# Autodesk Inventor assembly: Robot
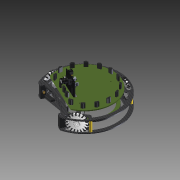
[picture p0: Inventor's stored thumbnail of the model, 180x180]
Saved by Autodesk Inventor 2015 (Build 190159000, 159)
## iProperties
Created: 2016-08-02
Part Number: Robot
Document SubType Name: Assembly
Designer: James Yelland
Author: James Yelland
## Documents named in this file (14)
- C:\Users\James Yelland\git\Layers-2017\Models\Robot.iam
- C:\Users\James Yelland\git\Layers-2017\Models\Bottom Plate.ipt
- C:\Users\James Yelland\git\Layers-2017\Models\Motor Mount.ipt
- C:\Users\James Yelland\git\Layers-2017\Models\Standoff 30.ipt
- C:\Users\James Yelland\git\Layers-2017\Models\Motor.ipt
- C:\Users\James Yelland\git\Layers-2017\Models\Middle Plate.ipt
- C:\Users\James Yelland\git\Layers-2017\Models\PCB.ipt
- C:\Users\James Yelland\git\Layers-2017\Models\Standoff 10.ipt
- C:\Users\James Yelland\git\Layers-2017\Models\Imported Components\Pixy(CMUcam5)\Pixy(CMUcam5).iam
- C:\Users\James Yelland\git\Layers-2017\Models\Light Sensor PCB.ipt
- C:\Users\James Yelland\git\Layers-2017\Models\Solenoid Mount.ipt
- C:\Users\James Yelland\git\Layers-2017\Models\Wheel.ipt
- C:\Users\James Yelland\git\Layers-2017\Models\Kicker Plate.ipt
- C:\Users\James Yelland\git\Layers-2017\Models\Laser Diode.ipt
## Components (24 placed, 13 different names)
1. Bottom Plate:1 — Mate:1, Mate:2, Mate:3, Mate:4, Mate:5, Mate:6, Mate:7, Mate:8, Mate:9, Mate:57, Mate:73, Mate:74, Mate:75, Mate:76, Mate:77, Mate:78, Mate:79, Mate:80, Mate:88, Mate:89, Mate:90, Flush:9, Flush:10
2. Motor Mount:1 — Mate:1, Mate:2, Mate:6, Mate:24, Mate:25, Mate:26
3. Motor Mount:2 — Mate:3, Mate:4, Mate:5, Mate:23, Mate:27, Mate:28
4. Motor Mount:3 — Mate:7, Mate:8, Mate:9, Mate:22, Mate:29, Mate:30
5. Motor:1 — Mate:24, Mate:25, Mate:26, Mate:91, Flush:7
6. Motor:2 — Mate:23, Mate:27, Mate:28, Mate:92, Flush:8
7. Motor:3 — Mate:22, Mate:29, Mate:30, Mate:93, Flush:6
8. Middle Plate:1 — Mate:37, Mate:38, Mate:39, Mate:40, Mate:41, Mate:42, Mate:87, Mate:94, Mate:98
9. PCB:1 — Mate:43, Mate:44, Mate:45, Mate:58, Mate:72
10. Standoff 10:1 — Mate:39, Mate:40, Mate:43
11. Standoff 10:2 — Mate:38, Mate:41, Mate:44
12. Standoff 10:3 — Mate:37, Mate:42, Mate:45
13. Pixy(CMUcam5):1 [sub-assembly] — Mate:57, Mate:58, Mate:72
14. Standoff 30:1 — Mate:79, Mate:80, Mate:87, Mate:94
15. Standoff 30:4 — Mate:77, Mate:78, Mate:98
16. Standoff 30:5 — Mate:75, Mate:76
17. Standoff 30:6 — Mate:73, Mate:74
18. Light Sensor PCB:1 — Mate:88, Mate:89
19. Solenoid Mount:1 — Mate:90, Flush:9, Flush:10, Mate:95, Mate:96, Mate:97, Mate:99, Flush:11
20. Wheel:1 — Mate:92, Flush:8
21. Wheel:2 — Mate:93, Flush:6
22. Wheel:3 — Mate:91, Flush:7
23. Kicker Plate:1 — Mate:95, Mate:96, Mate:97
24. Laser Diode:1 — Mate:99, Flush:11
## Relationships (57: Mate 51, Flush 6)
- Mate:1: Bottom Plate:1 ↔ Motor Mount:1
- Mate:2: Bottom Plate:1 ↔ Motor Mount:1
- Mate:3: Bottom Plate:1 ↔ Motor Mount:2
- Mate:4: Bottom Plate:1 ↔ Motor Mount:2
- Mate:5: Bottom Plate:1 ↔ Motor Mount:2
- Mate:6: Bottom Plate:1 ↔ Motor Mount:1
- Mate:7: Bottom Plate:1 ↔ Motor Mount:3
- Mate:8: Bottom Plate:1 ↔ Motor Mount:3
- Mate:9: Bottom Plate:1 ↔ Motor Mount:3
- Mate:22: Motor Mount:3 ↔ Motor:3
- Mate:23: Motor Mount:2 ↔ Motor:2
- Mate:24: Motor Mount:1 ↔ Motor:1
- Mate:25: Motor Mount:1 ↔ Motor:1
- Mate:26: Motor Mount:1 ↔ Motor:1
- Mate:27: Motor Mount:2 ↔ Motor:2
- Mate:28: Motor Mount:2 ↔ Motor:2
- Mate:29: Motor Mount:3 ↔ Motor:3
- Mate:30: Motor Mount:3 ↔ Motor:3
- Mate:37: Middle Plate:1 ↔ Standoff 10:3
- Mate:38: Middle Plate:1 ↔ Standoff 10:2
- Mate:39: Middle Plate:1 ↔ Standoff 10:1
- Mate:40: Middle Plate:1 ↔ Standoff 10:1
- Mate:41: Middle Plate:1 ↔ Standoff 10:2
- Mate:42: Middle Plate:1 ↔ Standoff 10:3
- Mate:43: PCB:1 ↔ Standoff 10:1
- Mate:44: PCB:1 ↔ Standoff 10:2
- Mate:45: PCB:1 ↔ Standoff 10:3
- Mate:57 (33 mm): Bottom Plate:1 ↔ Pixy(CMUcam5):1
- Mate:58 (3 mm): PCB:1 ↔ Pixy(CMUcam5):1
- Mate:72 (1 mm): PCB:1 ↔ Pixy(CMUcam5):1
- Mate:73: Bottom Plate:1 ↔ Standoff 30:6
- Mate:74: Bottom Plate:1 ↔ Standoff 30:6
- Mate:75: Bottom Plate:1 ↔ Standoff 30:5
- Mate:76: Bottom Plate:1 ↔ Standoff 30:5
- Mate:77: Bottom Plate:1 ↔ Standoff 30:4
- Mate:78: Bottom Plate:1 ↔ Standoff 30:4
- Mate:79: Bottom Plate:1 ↔ Standoff 30:1
- Mate:80: Bottom Plate:1 ↔ Standoff 30:1
- Mate:87: Middle Plate:1 ↔ Standoff 30:1
- Mate:88: Bottom Plate:1 ↔ Light Sensor PCB:1
- Mate:89: Bottom Plate:1 ↔ Light Sensor PCB:1
- Mate:90: Bottom Plate:1 ↔ Solenoid Mount:1
- Mate:91: Motor:1 ↔ Wheel:3
- Mate:92: Motor:2 ↔ Wheel:1
- Mate:93: Motor:3 ↔ Wheel:2
- Flush:6 (-6 mm): Motor:3 ↔ Wheel:2
- Flush:7 (-6 mm): Motor:1 ↔ Wheel:3
- Flush:8 (-6 mm): Motor:2 ↔ Wheel:1
- Mate:94: Middle Plate:1 ↔ Standoff 30:1
- Flush:9: Bottom Plate:1 ↔ Solenoid Mount:1
- Flush:10: Bottom Plate:1 ↔ Solenoid Mount:1
- Mate:95: Solenoid Mount:1 ↔ Kicker Plate:1
- Mate:96 (1 mm): Solenoid Mount:1 ↔ Kicker Plate:1
- Mate:97 (4.0075 mm): Solenoid Mount:1 ↔ Kicker Plate:1
- Mate:98: Middle Plate:1 ↔ Standoff 30:4
- Mate:99: Solenoid Mount:1 ↔ Laser Diode:1
- Flush:11 (-3 mm): Solenoid Mount:1 ↔ Laser Diode:1
